# Autodesk Inventor assembly: DriveUnit
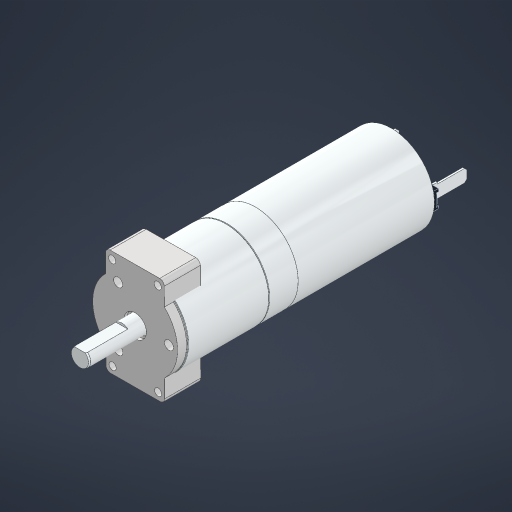
[picture p0: Inventor's stored thumbnail of the model, 512x512]
Saved by Autodesk Inventor 2024.2 (Build 282272000, 272)
## iProperties
Created: 2023-12-20
Part Number: DriveUnit
Document SubType Name: Assembly
Designer: Hanaoka
Author: Hanaoka
## Documents named in this file (4)
- G:\共有ドライブ\reRo\05_個人\hanaoka\inventor\DriveUnit.iam
- G:\共有ドライブ\reRo\05_個人\hanaoka\inventor\OmniWheel.iam
- G:\共有ドライブ\reRo\05_個人\hanaoka\inventor\Dcx19s_Gpx19c\Dcx19s_Gpx19c.iam
- G:\共有ドライブ\reRo\05_個人\hanaoka\inventor\MotorMount_sub.ipt
## Components (3 placed, 3 different names)
1. OmniWheel:1 [sub-assembly] — 挿入:1
2. Dcx19s_Gpx19c:1 [sub-assembly] — フラッシュ:1, フラッシュ:2, 正接:1, 挿入:1, 挿入:2
3. MotorMount_sub:1 — 挿入:2
## Relationships (5: Flush 2, Insert 2, Tangent 1)
- フラッシュ:1 [Flush]: Dcx19s_Gpx19c:1
- フラッシュ:2 [Flush] (-1.5 mm): Dcx19s_Gpx19c:1
- 正接:1 [Tangent] (-2 mm): Dcx19s_Gpx19c:1
- 挿入:1 [Insert]: OmniWheel:1 ↔ Dcx19s_Gpx19c:1
- 挿入:2 [Insert]: Dcx19s_Gpx19c:1 ↔ MotorMount_sub:1
